# Autodesk Inventor assembly: ElvShaft
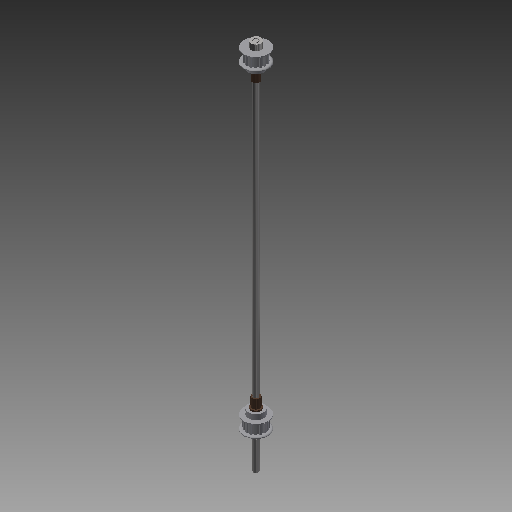
[picture p0: Inventor's stored thumbnail of the model, 512x512]
Saved by Autodesk Inventor 2019 (Build 230136000, 136)
## iProperties
Created: 2019-01-10
Part Number: ElvShaft
Document SubType Name: Assembly
Designer: james
Mass: 179.45 g
Surface Area: 167.573 cm^2
Volume: 22.4285 cm^3
Density: 8.00099 g/cm^3
Author: james
## Documents named in this file (5)
- F:\JimsDesign\2019CHS4089\ElvShaft.iam
- F:\JimsDesign\Library\McMaster\1327K670_MINIATURE 12L14 DRIVE STEEL SHAFT.ipt
- F:\JimsDesign\Library\McMaster\9414T600_SET SCREW SHAFT COLLAR.ipt
- F:\JimsDesign\Library\McMaster\6338K413_OIL-EMBEDDED FLANGED SLEEVE BEARING.ipt
- F:\JimsDesign\Library\McMaster\57105K150_XL SERIES LIGHTWEIGHT TIMING BELT PULLEY.ipt
## Components (7 placed, 4 different names)
1. 1327K670_MINIATURE 12L14 DRIVE STEEL SHAFT:1 — Mate:1, Flush:1, Mate:2, Flush:2, Mate:7, Mate:9, Mate:11, Mate:14
2. 9414T600_SET SCREW SHAFT COLLAR:1 — Mate:1, Flush:1, Mate:15
3. 9414T600_SET SCREW SHAFT COLLAR:2 — Mate:2, Flush:2, Mate:10
4. 57105K150_XL SERIES LIGHTWEIGHT TIMING BELT PULLEY:1 — Mate:10, Mate:11, Mate:12
5. 57105K150_XL SERIES LIGHTWEIGHT TIMING BELT PULLEY:2 — Mate:13, Mate:14, Mate:15
6. 6338K413_OIL-EMBEDDED FLANGED SLEEVE BEARING:1 — Mate:9, Mate:13
7. 6338K413_OIL-EMBEDDED FLANGED SLEEVE BEARING:2 — Mate:7, Mate:12
## Relationships (12: Mate 10, Flush 2)
- Mate:1: 1327K670_MINIATURE 12L14 DRIVE STEEL SHAFT:1 ↔ 9414T600_SET SCREW SHAFT COLLAR:1
- Flush:1 (-38.1 mm): 1327K670_MINIATURE 12L14 DRIVE STEEL SHAFT:1 ↔ 9414T600_SET SCREW SHAFT COLLAR:1
- Mate:2: 1327K670_MINIATURE 12L14 DRIVE STEEL SHAFT:1 ↔ 9414T600_SET SCREW SHAFT COLLAR:2
- Flush:2: 1327K670_MINIATURE 12L14 DRIVE STEEL SHAFT:1 ↔ 9414T600_SET SCREW SHAFT COLLAR:2
- Mate:7: 1327K670_MINIATURE 12L14 DRIVE STEEL SHAFT:1 ↔ 6338K413_OIL-EMBEDDED FLANGED SLEEVE BEARING:2
- Mate:9: 1327K670_MINIATURE 12L14 DRIVE STEEL SHAFT:1 ↔ 6338K413_OIL-EMBEDDED FLANGED SLEEVE BEARING:1
- Mate:10: 9414T600_SET SCREW SHAFT COLLAR:2 ↔ 57105K150_XL SERIES LIGHTWEIGHT TIMING BELT PULLEY:1
- Mate:11: 1327K670_MINIATURE 12L14 DRIVE STEEL SHAFT:1 ↔ 57105K150_XL SERIES LIGHTWEIGHT TIMING BELT PULLEY:1
- Mate:12: 57105K150_XL SERIES LIGHTWEIGHT TIMING BELT PULLEY:1 ↔ 6338K413_OIL-EMBEDDED FLANGED SLEEVE BEARING:2
- Mate:13: 57105K150_XL SERIES LIGHTWEIGHT TIMING BELT PULLEY:2 ↔ 6338K413_OIL-EMBEDDED FLANGED SLEEVE BEARING:1
- Mate:14: 1327K670_MINIATURE 12L14 DRIVE STEEL SHAFT:1 ↔ 57105K150_XL SERIES LIGHTWEIGHT TIMING BELT PULLEY:2
- Mate:15: 9414T600_SET SCREW SHAFT COLLAR:1 ↔ 57105K150_XL SERIES LIGHTWEIGHT TIMING BELT PULLEY:2
